# Autodesk Inventor assembly: Broncos Assembly3
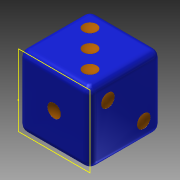
[picture p0: Inventor's stored thumbnail of the model, 180x180]
Saved by Autodesk Inventor 2014 (Build 180170000, 170)
## iProperties
Created: 2013-09-03
Part Number: Broncos Assembly3
Document SubType Name: Assembly
Designer: s601298
Author: s601298
## Documents named in this file (3)
- C:\Quinn\Grabcad\Dice\Broncos\Broncos Assembly.iam
- C:\Quinn\Grabcad\Dice\Broncos\Broncos.ipt
- C:\Quinn\Grabcad\Dice\Broncos\OrangePip.ipt
## Components (22 placed, 2 different names)
1. Broncos:1 — Insert:1, Insert:2, Insert:3, Insert:4, Insert:5, Insert:6, Insert:7, Insert:8, Insert:9, Insert:10, Insert:11, Insert:12, Insert:13, Insert:14, Insert:15, Insert:16, Insert:17, Insert:18, Insert:19, Insert:20, Insert:21
2. OrangePip:1 — Insert:16
3. OrangePip:2 — Insert:17
4. OrangePip:3 — Insert:21
5. OrangePip:4 — Insert:20
6. OrangePip:5 — Insert:19
7. OrangePip:6 — Insert:18
8. OrangePip:7 — Insert:15
9. OrangePip:8 — Insert:14
10. OrangePip:9 — Insert:11
11. OrangePip:10 — Insert:9
12. OrangePip:11 — Insert:8
13. OrangePip:12 — Insert:13
14. OrangePip:13 — Insert:12
15. OrangePip:14 — Insert:10
16. OrangePip:15 — Insert:7
17. OrangePip:16 — Insert:6
18. OrangePip:17 — Insert:4
19. OrangePip:18 — Insert:5
20. OrangePip:19 — Insert:1
21. OrangePip:20 — Insert:2
22. OrangePip:21 — Insert:3
## Relationships (21: Insert 21)
- Insert:1: Broncos:1 ↔ OrangePip:19
- Insert:2: Broncos:1 ↔ OrangePip:20
- Insert:3: Broncos:1 ↔ OrangePip:21
- Insert:4: Broncos:1 ↔ OrangePip:17
- Insert:5: Broncos:1 ↔ OrangePip:18
- Insert:6: Broncos:1 ↔ OrangePip:16
- Insert:7: Broncos:1 ↔ OrangePip:15
- Insert:8: Broncos:1 ↔ OrangePip:11
- Insert:9: Broncos:1 ↔ OrangePip:10
- Insert:10: Broncos:1 ↔ OrangePip:14
- Insert:11: Broncos:1 ↔ OrangePip:9
- Insert:12: Broncos:1 ↔ OrangePip:13
- Insert:13: Broncos:1 ↔ OrangePip:12
- Insert:14: Broncos:1 ↔ OrangePip:8
- Insert:15: Broncos:1 ↔ OrangePip:7
- Insert:16: Broncos:1 ↔ OrangePip:1
- Insert:17: Broncos:1 ↔ OrangePip:2
- Insert:18: Broncos:1 ↔ OrangePip:6
- Insert:19: Broncos:1 ↔ OrangePip:5
- Insert:20: Broncos:1 ↔ OrangePip:4
- Insert:21: Broncos:1 ↔ OrangePip:3
